# Autodesk Inventor assembly: RIGHT FRAME
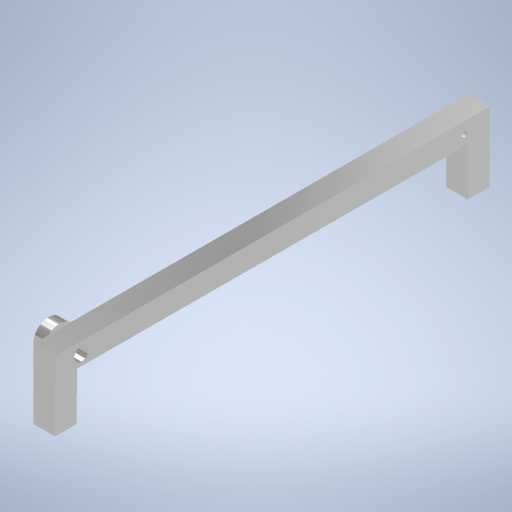
[picture p0: Inventor's stored thumbnail of the model, 512x512]
Saved by Autodesk Inventor 2023 (Build 270158000, 158)
## iProperties
Created: 2022-08-29
Part Number: RIGHT FRAME
Document SubType Name: Assembly
Designer: D.C. Eksteen
Author: D.C. Eksteen
Title: RIGHT REAR FRAME ASSEMBLY
## Documents named in this file (5)
- C:\Users\dylan\Desktop\Skripsie-2022\Design\CAD\RIGHT FRAME.iam
- C:\Users\dylan\Desktop\Skripsie-2022\Design\CAD\RIGHT TOP TUBE.ipt
- C:\Users\dylan\Desktop\Skripsie-2022\Design\CAD\RISER.ipt
- C:\Users\dylan\Desktop\Skripsie-2022\Design\CAD\BEARING BLOCK.ipt
- C:\Users\dylan\Desktop\Skripsie-2022\Design\CAD\472-028.ipt
## Components (5 placed, 4 different names)
1. RIGHT TOP TUBE:1 — Mate:1, Flush:1, Mate:2, Flush:2, Mate:3, Mate:4, Mate:10, Mate:16
2. RISER:1 — Mate:1, Flush:1, Mate:4
3. RISER:2 — Mate:2, Flush:2, Mate:3
4. BEARING BLOCK:1 — Mate:10, Mate:12, Mate:13, Mate:16
5. UNI 7437 28:1 — Mate:12, Mate:13
## Relationships (10: Mate 8, Flush 2)
- Mate:1: RIGHT TOP TUBE:1 ↔ RISER:1
- Flush:1: RIGHT TOP TUBE:1 ↔ RISER:1
- Mate:2: RIGHT TOP TUBE:1 ↔ RISER:2
- Flush:2: RIGHT TOP TUBE:1 ↔ RISER:2
- Mate:3: RIGHT TOP TUBE:1 ↔ RISER:2
- Mate:4: RIGHT TOP TUBE:1 ↔ RISER:1
- Mate:10: RIGHT TOP TUBE:1 ↔ BEARING BLOCK:1
- Mate:12: BEARING BLOCK:1 ↔ UNI 7437 28:1
- Mate:13: BEARING BLOCK:1 ↔ UNI 7437 28:1
- Mate:16: RIGHT TOP TUBE:1 ↔ BEARING BLOCK:1
